# Autodesk Inventor assembly: 276-1447-002
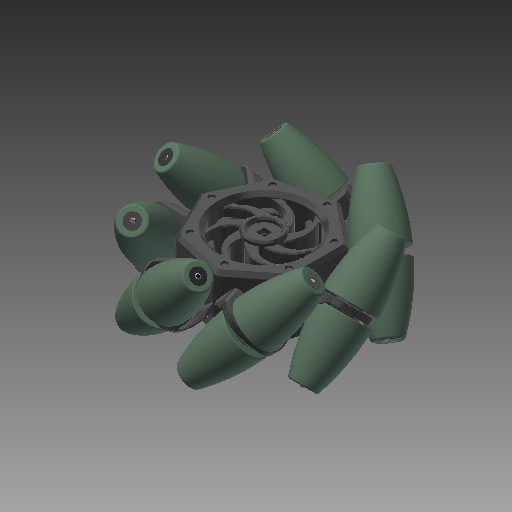
[picture p0: Inventor's stored thumbnail of the model, 512x512]
Saved by Autodesk Inventor 2019 (Build 230136000, 136)
## iProperties
Company: Bots 'n' Stuff Robotics
Created: 2011-11-15
Part Number: 276-1447-002
Document SubType Name: Assembly
Designer: Jordan Kiesel
Catalog Web Link: http://www.vexrobotics.com/276-1447.html
Vendor: VEX Robotics, Inc.
Author: Jordan Kiesel
Title: 4" Mecanum Wheel - Right
## Documents named in this file (8)
- C:\Users\Lazo Attar\Documents\GitHub\carnegie285XCAD\2018 BNS-VRC-SID Library\Motion\Wheels _ Rollers\4_ Mecanum Wheel - Right.iam
- C:\Users\Lazo Attar\Documents\GitHub\carnegie285XCAD\2018 BNS-VRC-SID Library\Motion\Wheels _ Rollers\Reference Parts\Mecanum Wheels\Washer.ipt
- C:\Users\Lazo Attar\Documents\GitHub\carnegie285XCAD\2018 BNS-VRC-SID Library\Motion\Wheels _ Rollers\Reference Parts\Mecanum Wheels\Small Wheel Hub.ipt
- C:\Users\Lazo Attar\Documents\GitHub\carnegie285XCAD\2018 BNS-VRC-SID Library\Motion\Wheels _ Rollers\Reference Parts\Mecanum Wheels\Pin.ipt
- C:\Users\Lazo Attar\Documents\GitHub\carnegie285XCAD\2018 BNS-VRC-SID Library\Motion\Wheels _ Rollers\Reference Parts\Mecanum Wheels\Wheel.ipt
- C:\Users\Lazo Attar\Documents\GitHub\carnegie285XCAD\2018 BNS-VRC-SID Library\Motion\Wheels _ Rollers\Reference Parts\Mecanum Wheels\Wheel Hub Out R.ipt
- C:\Users\Lazo Attar\Documents\GitHub\carnegie285XCAD\2018 BNS-VRC-SID Library\Motion\Wheels _ Rollers\Reference Parts\Mecanum Wheels\Wheel Hub In R.ipt
- C:\Users\Lazo Attar\Documents\GitHub\carnegie285XCAD\2018 BNS-VRC-SID Library\Motion\Wheels _ Rollers\Reference Parts\Mecanum Wheels\Bracket R.ipt
## Components (58 placed, 7 different names)
1. Wheel Hub Out R:1 — Mate:1, Mate:2, Mate:3, Mate:4, Mate:5, Mate:6, Mate:7, Mate:8, Mate:9, Mate:10, Mate:11, Mate:12, Mate:13, Mate:14, Mate:15, Mate:16, Mate:17, Mate:18, Mate:19, Mate:20, Mate:21, Mate:22, Mate:23, Mate:24
2. Bracket R:1 — Mate:1, Mate:2, Mate:3, Insert:1, Insert:2
3. Bracket R:2 — Mate:7, Mate:8, Mate:9, Insert:3, Insert:4
4. Bracket R:3 — Mate:10, Mate:11, Mate:12, Insert:5, Insert:6
5. Bracket R:4 — Mate:13, Mate:14, Mate:15, Insert:7, Insert:8
6. Bracket R:5 — Mate:16, Mate:17, Mate:18, Insert:9, Insert:10
7. Bracket R:6 — Mate:19, Mate:20, Mate:21, Insert:11, Insert:12
8. Bracket R:7 — Mate:22, Mate:23, Mate:24, Insert:13, Insert:14
9. Wheel Hub In R:1 — Mate:4, Mate:5, Mate:6
10. Washer:1 — Insert:1, Insert:15
11. Washer:2 — Insert:2, Insert:16
12. Washer:3 — Insert:3, Insert:17
13. Washer:4 — Insert:4, Insert:18
14. Washer:5 — Insert:5, Insert:19
15. Washer:6 — Insert:6, Insert:20
16. Washer:7 — Insert:7, Insert:21
17. Washer:8 — Insert:8, Insert:22
18. Washer:9 — Insert:9, Insert:23
19. Washer:10 — Insert:10, Insert:24
20. Washer:11 — Insert:11, Insert:25
21. Washer:12 — Insert:12, Insert:26
22. Washer:13 — Insert:13, Insert:27
23. Washer:14 — Insert:14, Insert:28
24. Small Wheel Hub:1 — Insert:15, Insert:29, Insert:36
25. Small Wheel Hub:2 — Insert:16, Insert:37
26. Small Wheel Hub:3 — Insert:17, Insert:30, Insert:38
27. Small Wheel Hub:4 — Insert:18, Insert:39
28. Small Wheel Hub:5 — Insert:19, Insert:31, Insert:40
29. Small Wheel Hub:6 — Insert:20, Insert:41
30. Small Wheel Hub:7 — Insert:21, Insert:32, Insert:42
31. Small Wheel Hub:8 — Insert:22, Insert:43
32. Small Wheel Hub:9 — Insert:23, Insert:33, Insert:44
33. Small Wheel Hub:10 — Insert:24, Insert:45
34. Small Wheel Hub:11 — Insert:25, Insert:34, Insert:46
35. Small Wheel Hub:12 — Insert:26, Insert:47
36. Small Wheel Hub:13 — Insert:27, Insert:35, Insert:48
37. Small Wheel Hub:14 — Insert:28, Insert:49
38. Pin:1 — Insert:29
39. Pin:2 — Insert:30
40. Pin:3 — Insert:31
41. Pin:4 — Insert:32
42. Pin:5 — Insert:33
43. Pin:6 — Insert:34
44. Pin:7 — Insert:35
45. Wheel:1 — Insert:36
46. Wheel:2 — Insert:37
47. Wheel:3 — Insert:38
48. Wheel:4 — Insert:39
49. Wheel:5 — Insert:40
50. Wheel:6 — Insert:41
51. Wheel:7 — Insert:42
52. Wheel:8 — Insert:43
53. Wheel:9 — Insert:44
54. Wheel:10 — Insert:45
55. Wheel:11 — Insert:46
56. Wheel:12 — Insert:47
57. Wheel:13 — Insert:48
58. Wheel:14 — Insert:49
## Relationships (73: Insert 49, Mate 24)
- Mate:1 (0.05 mm): Wheel Hub Out R:1 ↔ Bracket R:1
- Mate:2 (0.0542 mm): Wheel Hub Out R:1 ↔ Bracket R:1
- Mate:3 (0.1317 mm): Wheel Hub Out R:1 ↔ Bracket R:1
- Mate:4: Wheel Hub Out R:1 ↔ Wheel Hub In R:1
- Mate:5: Wheel Hub Out R:1 ↔ Wheel Hub In R:1
- Mate:6: Wheel Hub Out R:1 ↔ Wheel Hub In R:1
- Mate:7 (0.05 mm): Wheel Hub Out R:1 ↔ Bracket R:2
- Mate:8 (0.0542 mm): Wheel Hub Out R:1 ↔ Bracket R:2
- Mate:9 (0.1317 mm): Wheel Hub Out R:1 ↔ Bracket R:2
- Mate:10 (0.05 mm): Wheel Hub Out R:1 ↔ Bracket R:3
- Mate:11 (0.0542 mm): Wheel Hub Out R:1 ↔ Bracket R:3
- Mate:12 (0.1317 mm): Wheel Hub Out R:1 ↔ Bracket R:3
- Mate:13 (0.05 mm): Wheel Hub Out R:1 ↔ Bracket R:4
- Mate:14 (0.0542 mm): Wheel Hub Out R:1 ↔ Bracket R:4
- Mate:15 (0.1317 mm): Wheel Hub Out R:1 ↔ Bracket R:4
- Mate:16 (0.05 mm): Wheel Hub Out R:1 ↔ Bracket R:5
- Mate:17 (0.0542 mm): Wheel Hub Out R:1 ↔ Bracket R:5
- Mate:18 (0.1317 mm): Wheel Hub Out R:1 ↔ Bracket R:5
- Mate:19 (0.05 mm): Wheel Hub Out R:1 ↔ Bracket R:6
- Mate:20 (0.0542 mm): Wheel Hub Out R:1 ↔ Bracket R:6
- Mate:21 (0.1317 mm): Wheel Hub Out R:1 ↔ Bracket R:6
- Mate:22 (0.05 mm): Wheel Hub Out R:1 ↔ Bracket R:7
- Mate:23 (0.0542 mm): Wheel Hub Out R:1 ↔ Bracket R:7
- Mate:24 (0.1317 mm): Wheel Hub Out R:1 ↔ Bracket R:7
- Insert:1: Bracket R:1 ↔ Washer:1
- Insert:2: Bracket R:1 ↔ Washer:2
- Insert:3: Bracket R:2 ↔ Washer:3
- Insert:4: Bracket R:2 ↔ Washer:4
- Insert:5: Bracket R:3 ↔ Washer:5
- Insert:6: Bracket R:3 ↔ Washer:6
- Insert:7: Bracket R:4 ↔ Washer:7
- Insert:8: Bracket R:4 ↔ Washer:8
- Insert:9: Bracket R:5 ↔ Washer:9
- Insert:10: Bracket R:5 ↔ Washer:10
- Insert:11: Bracket R:6 ↔ Washer:11
- Insert:12: Bracket R:6 ↔ Washer:12
- Insert:13: Bracket R:7 ↔ Washer:13
- Insert:14: Bracket R:7 ↔ Washer:14
- Insert:15: Washer:1 ↔ Small Wheel Hub:1
- Insert:16: Washer:2 ↔ Small Wheel Hub:2
- Insert:17: Washer:3 ↔ Small Wheel Hub:3
- Insert:18: Washer:4 ↔ Small Wheel Hub:4
- Insert:19: Washer:5 ↔ Small Wheel Hub:5
- Insert:20: Washer:6 ↔ Small Wheel Hub:6
- Insert:21: Washer:7 ↔ Small Wheel Hub:7
- Insert:22: Washer:8 ↔ Small Wheel Hub:8
- Insert:23: Washer:9 ↔ Small Wheel Hub:9
- Insert:24: Washer:10 ↔ Small Wheel Hub:10
- Insert:25: Washer:11 ↔ Small Wheel Hub:11
- Insert:26: Washer:12 ↔ Small Wheel Hub:12
- Insert:27: Washer:13 ↔ Small Wheel Hub:13
- Insert:28: Washer:14 ↔ Small Wheel Hub:14
- Insert:29 (-0.5001 mm): Small Wheel Hub:1 ↔ Pin:1
- Insert:30 (-0.5001 mm): Small Wheel Hub:3 ↔ Pin:2
- Insert:31 (-0.5001 mm): Small Wheel Hub:5 ↔ Pin:3
- Insert:32 (-0.5001 mm): Small Wheel Hub:7 ↔ Pin:4
- Insert:33 (-0.5001 mm): Small Wheel Hub:9 ↔ Pin:5
- Insert:34 (-0.5001 mm): Small Wheel Hub:11 ↔ Pin:6
- Insert:35 (-0.5001 mm): Small Wheel Hub:13 ↔ Pin:7
- Insert:36: Small Wheel Hub:1 ↔ Wheel:1
- Insert:37: Small Wheel Hub:2 ↔ Wheel:2
- Insert:38: Small Wheel Hub:3 ↔ Wheel:3
- Insert:39: Small Wheel Hub:4 ↔ Wheel:4
- Insert:40: Small Wheel Hub:5 ↔ Wheel:5
- Insert:41: Small Wheel Hub:6 ↔ Wheel:6
- Insert:42: Small Wheel Hub:7 ↔ Wheel:7
- Insert:43: Small Wheel Hub:8 ↔ Wheel:8
- Insert:44: Small Wheel Hub:9 ↔ Wheel:9
- Insert:45: Small Wheel Hub:10 ↔ Wheel:10
- Insert:46: Small Wheel Hub:11 ↔ Wheel:11
- Insert:47: Small Wheel Hub:12 ↔ Wheel:12
- Insert:48: Small Wheel Hub:13 ↔ Wheel:13
- Insert:49: Small Wheel Hub:14 ↔ Wheel:14
## Named parameters: offset1 = 0.05 mm, offset2 = 0.05423 mm, max2 = 0.10847 mm, min2 = 0 mm, max1 = 0.1 mm, min1 = 0 mm, offset3 = 0.1317 mm, max3 = 0.2634 mm, min3 = 0 mm, offset4 = -0.50011 mm
